# Autodesk Inventor assembly: Micro_CNC
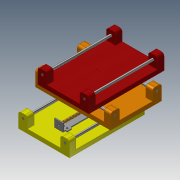
[picture p0: Inventor's stored thumbnail of the model, 180x180]
Saved by Autodesk Inventor 2014 SP1 (Build 180222100, 222)
## iProperties
Created: 2014-03-24
Part Number: Micro_CNC
Document SubType Name: Assembly
Designer: tom
Author: tom
## Documents named in this file (5)
- C:\Users\tom\Documents\GitHub\Micro_CNC\Inventor Models\Micro_CNC.iam
- C:\Users\tom\Documents\GitHub\Micro_CNC\Inventor Models\Motor.iam
- C:\Users\tom\Documents\GitHub\Micro_CNC\Inventor Models\Base1.ipt
- C:\Users\tom\Documents\GitHub\Micro_CNC\Inventor Models\Shaft.ipt
- C:\Users\tom\Documents\GitHub\Boat_Bot\Middle Carriage.iam
## Components (6 placed, 5 different names)
1. Motor:1 [sub-assembly] — Mate:1
2. Base1:1 — Mate:1, Mate:2, Mate:3, Mate:4
3. Shaft:1 — Mate:2, Mate:3
4. Shaft:2 — Mate:4
5. Middle Carriage [sub-assembly] — Cylindrical:3, Cylindrical:4
6. Top Carriage [sub-assembly] — Cylindrical:3, Cylindrical:4
## Relationships (8: Mate 4, CylindricalJoint 4)
- Mate:1: Motor:1 ↔ Base1:1
- Mate:2: Base1:1 ↔ Shaft:1
- [CylindricalJoint]: Shaft:2 ↔ Middle Carriage
- [CylindricalJoint]: Shaft:1 ↔ Middle Carriage
- Mate:3: Base1:1 ↔ Shaft:1
- Mate:4: Base1:1 ↔ Shaft:2
- Cylindrical:3: Middle Carriage ↔ Top Carriage
- Cylindrical:4: Middle Carriage ↔ Top Carriage
